# Autodesk Inventor assembly: end-support-assembly-parts
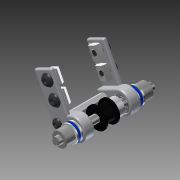
[picture p0: Inventor's stored thumbnail of the model, 180x180]
Saved by Autodesk Inventor 2015 (Build 190159000, 159)
## iProperties
Created: 2013-07-07
Part Number: end-support-assembly-parts
Document SubType Name: Assembly
Designer: mhgreen
Author: mhgreen
## Documents named in this file (12)
- C:\Users\Michael\Documents\GitHub\openbuilds-parts\example assemblies\end support assembly\end-support-assembly-parts.iam
- C:\Users\Michael\Documents\GitHub\openbuilds-parts\example assemblies\end support assembly\13mmBearingBracketLeft.ipt
- C:\Users\Michael\Documents\GitHub\openbuilds-parts\example assemblies\end support assembly\13mmBearingBracketRight.ipt
- C:\Users\Michael\Documents\GitHub\openbuilds-parts\example assemblies\end support assembly\Bearing_6x13x5_a_7y_5mpss1306.ipt
- C:\Users\Michael\Documents\GitHub\openbuilds-parts\example assemblies\end support assembly\6mmThrust_a_7z_7m0614st.ipt
- C:\Users\Michael\Documents\GitHub\openbuilds-parts\example assemblies\end support assembly\6mmShaftCollar_a_7c_2m112060.ipt
- C:\Users\Michael\Documents\GitHub\openbuilds-parts\example assemblies\end support assembly\M4_30MM_95947A062.ipt
- C:\Users\Michael\Documents\GitHub\openbuilds-parts\example assemblies\end support assembly\80mm shaft.ipt
- C:\Users\Michael\Documents\GitHub\openbuilds-parts\example assemblies\end support assembly\MXL20T6MMbore6T16M020DF6006.ipt
- C:\Users\Michael\Documents\GitHub\openbuilds-parts\example assemblies\end support assembly\HNTT5_5.ipt
- C:\Users\Michael\Documents\GitHub\openbuilds-parts\example assemblies\end support assembly\91239A222.ipt
- C:\Users\Michael\Documents\GitHub\openbuilds-parts\example assemblies\end support assembly\91239A150.ipt
## Components (24 placed, 11 different names)
1. 13mmBearingBracketLeft:1 — Insert:1, Mate:7, Insert:12, Insert:13, Insert:16, Insert:17, Angle:5, Angle:6, Insert:24, Insert:25
2. 13mmBearingBracketRight:1 — Insert:2, Insert:6, Insert:8, Insert:9, Insert:14, Insert:15, Angle:3, Angle:4, Insert:22, Insert:23
3. Bearing_6x13x5_a_7y_5mpss1306:1 — Insert:2
4. Bearing_6x13x5_a_7y_5mpss1306:2 — Insert:1
5. 6mmThrust_a_7z_7m0614st:1 — Insert:6, Insert:7
6. 6mmThrust_a_7z_7m0614st:2 — Mate:7, Insert:5
7. 6mmShaftCollar_a_7c_2m112060:1 — Insert:5, Insert:10
8. 6mmShaftCollar_a_7c_2m112060:2 — Insert:7
9. M4_30MM_95947A062:1 — Insert:8, Insert:13
10. M4_30MM_95947A062:2 — Insert:9, Insert:12
11. 80mm shaft:1 — Insert:10, Insert:11
12. MXL20T6MMbore6T16M020DF6006:1 — Insert:11
13. HNTT5_5:1 — Insert:18, Angle:5
14. HNTT5_5:2 — Insert:19, Angle:6
15. HNTT5_5:3 — Insert:20, Angle:4
16. HNTT5_5:4 — Insert:21, Angle:3
17. 91239A222:1 — Insert:17, Insert:19
18. 91239A222:2 — Insert:15, Insert:20
19. 91239A222:3 — Insert:14, Insert:21
20. 91239A222:4 — Insert:16, Insert:18
21. 91239A150:1 — Insert:24
22. 91239A150:2 — Insert:25
23. 91239A150:3 — Insert:23
24. 91239A150:4 — Insert:22
## Relationships (28: Insert 23, Angle 4, Mate 1)
- Insert:1: 13mmBearingBracketLeft:1 ↔ Bearing_6x13x5_a_7y_5mpss1306:2
- Insert:2: 13mmBearingBracketRight:1 ↔ Bearing_6x13x5_a_7y_5mpss1306:1
- Mate:7: 13mmBearingBracketLeft:1 ↔ 6mmThrust_a_7z_7m0614st:2
- Insert:5: 6mmThrust_a_7z_7m0614st:2 ↔ 6mmShaftCollar_a_7c_2m112060:1
- Insert:6: 13mmBearingBracketRight:1 ↔ 6mmThrust_a_7z_7m0614st:1
- Insert:7: 6mmThrust_a_7z_7m0614st:1 ↔ 6mmShaftCollar_a_7c_2m112060:2
- Insert:8: 13mmBearingBracketRight:1 ↔ M4_30MM_95947A062:1
- Insert:9: 13mmBearingBracketRight:1 ↔ M4_30MM_95947A062:2
- Insert:10 (-3.2 mm): 6mmShaftCollar_a_7c_2m112060:1 ↔ 80mm shaft:1
- Insert:11 (-45.5 mm): 80mm shaft:1 ↔ MXL20T6MMbore6T16M020DF6006:1
- Insert:12: 13mmBearingBracketLeft:1 ↔ M4_30MM_95947A062:2
- Insert:13: 13mmBearingBracketLeft:1 ↔ M4_30MM_95947A062:1
- Insert:14: 13mmBearingBracketRight:1 ↔ 91239A222:3
- Insert:15: 13mmBearingBracketRight:1 ↔ 91239A222:2
- Insert:16: 13mmBearingBracketLeft:1 ↔ 91239A222:4
- Insert:17: 13mmBearingBracketLeft:1 ↔ 91239A222:1
- Insert:18: HNTT5_5:1 ↔ 91239A222:4
- Insert:19: HNTT5_5:2 ↔ 91239A222:1
- Insert:20: HNTT5_5:3 ↔ 91239A222:2
- Insert:21: HNTT5_5:4 ↔ 91239A222:3
- Angle:3 (90 deg): 13mmBearingBracketRight:1 ↔ HNTT5_5:4
- Angle:4 (90 deg): 13mmBearingBracketRight:1 ↔ HNTT5_5:3
- Angle:5 (90 deg): 13mmBearingBracketLeft:1 ↔ HNTT5_5:1
- Angle:6 (90 deg): 13mmBearingBracketLeft:1 ↔ HNTT5_5:2
- Insert:22: 13mmBearingBracketRight:1 ↔ 91239A150:4
- Insert:23: 13mmBearingBracketRight:1 ↔ 91239A150:3
- Insert:24: 13mmBearingBracketLeft:1 ↔ 91239A150:1
- Insert:25: 13mmBearingBracketLeft:1 ↔ 91239A150:2
